# Autodesk Inventor assembly: WheelIntake4.0
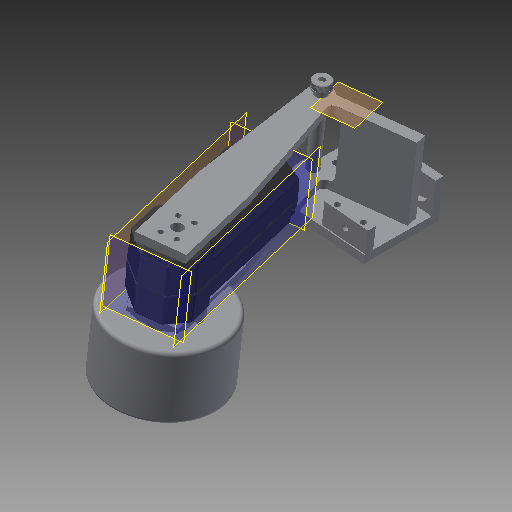
[picture p0: Inventor's stored thumbnail of the model, 512x512]
Saved by Autodesk Inventor 2019 (Build 230136000, 136)
## iProperties
Created: 2017-12-13
Part Number: WheelIntake4.0
Document SubType Name: Assembly
Designer: User
Author: User
## Documents named in this file (7)
- C:\Robotics\CAD\2017-18_CAD\WheelIntake5.0.iam
- C:\Robotics\CAD\COTSParts\Rev\REV-41-1300HexMotor.ipt
- C:\Robotics\CAD\COTSParts\Fasteners\97345A171_TYPE 316 STAINLESS STEEL SHOULDER SCREW.ipt
- C:\Robotics\CAD\COTSParts\Wheels\2.5inFoamWheel250TMD.ipt
- C:\Robotics\CAD\2017-18_CAD\WheelIntake5.0Base.ipt
- C:\Robotics\CAD\2017-18_CAD\WheelIntake5.0Mount.ipt
- C:\Robotics\CAD\2017-18_CAD\WheelIntakeSpringStop.ipt
## Components (6 placed, 6 different names)
1. REV-41-1300HexMotor:1 — Insert:2, Insert:3
2. 97345A171_TYPE 316 STAINLESS STEEL SHOULDER SCREW:1 — Insert:1, Insert:8
3. 2.5inFoamWheel250TMD:1 — Insert:7
4. WheelIntake5.0Base:1 — Insert:8, Insert:9, Insert:10
5. WheelIntake5.0Mount:1 — Insert:1, Insert:2, Insert:3, Insert:7
6. WheelIntakeSpringStop:1 — Insert:9, Insert:10
## Relationships (7: Insert 7)
- Insert:1: 97345A171_TYPE 316 STAINLESS STEEL SHOULDER SCREW:1 ↔ WheelIntake5.0Mount:1
- Insert:2: REV-41-1300HexMotor:1 ↔ WheelIntake5.0Mount:1
- Insert:3: REV-41-1300HexMotor:1 ↔ WheelIntake5.0Mount:1
- Insert:7: 2.5inFoamWheel250TMD:1 ↔ WheelIntake5.0Mount:1
- Insert:8: 97345A171_TYPE 316 STAINLESS STEEL SHOULDER SCREW:1 ↔ WheelIntake5.0Base:1
- Insert:9: WheelIntake5.0Base:1 ↔ WheelIntakeSpringStop:1
- Insert:10: WheelIntake5.0Base:1 ↔ WheelIntakeSpringStop:1
